# Autodesk Inventor assembly: Terminal Connector
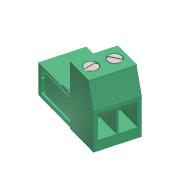
[picture p0: Inventor's stored thumbnail of the model, 180x180]
Saved by Autodesk Inventor 2022 (Build 260153000, 153)
## iProperties
Created: 2019-08-19
Part Number: Terminal Connector
Document SubType Name: Assembly
Designer: SENSE IT OUT
Author: SENSE IT OUT
## Documents named in this file (4)
- C:\Users\ferna\Downloads\pluggable-terminal-connector-2-pin-1.snapshot.1\Terminal Connector.iam
- C:\Users\ferna\Downloads\pluggable-terminal-connector-2-pin-1.snapshot.1\Plugin_block.ipt
- C:\Users\ferna\Downloads\pluggable-terminal-connector-2-pin-1.snapshot.1\plugin_maleblock.ipt
- C:\Users\ferna\Downloads\pluggable-terminal-connector-2-pin-1.snapshot.1\Screw_Terminal.ipt
## Components (4 placed, 3 different names)
1. Plugin_block:1 — Mate:1, Mate:2, Flush:1, Mate:3, Mate:4, Mate:5, Mate:6
2. plugin_maleblock:1 — Mate:1, Mate:2, Flush:1
3. Screw_Terminal:1 — Mate:3, Mate:6
4. Screw_Terminal:2 — Mate:4, Mate:5
## Relationships (7: Mate 6, Flush 1)
- Mate:1: Plugin_block:1 ↔ plugin_maleblock:1
- Mate:2: Plugin_block:1 ↔ plugin_maleblock:1
- Flush:1: Plugin_block:1 ↔ plugin_maleblock:1
- Mate:3: Plugin_block:1 ↔ Screw_Terminal:1
- Mate:4: Plugin_block:1 ↔ Screw_Terminal:2
- Mate:5: Plugin_block:1 ↔ Screw_Terminal:2
- Mate:6: Plugin_block:1 ↔ Screw_Terminal:1
